# Autodesk Inventor assembly: Rod
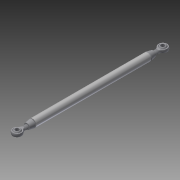
[picture p0: Inventor's stored thumbnail of the model, 180x180]
Saved by Autodesk Inventor 2015 (Build 190159000, 159)
## iProperties
Created: 2016-04-07
Part Number: Rod
Document SubType Name: Assembly
Designer: Mac
Author: Mac
## Documents named in this file (4)
- C:\Users\Mac\Desktop\MotionBase\CAD\MotionBaseCAD\Real Platform\Rod.iam
- C:\Users\Mac\Desktop\MotionBase\CAD\MotionBaseCAD\Real Platform\Rod.ipt
- C:\Users\Mac\Desktop\MotionBase\CAD\MotionBaseCAD\Real Platform\BallJoint.ipt
- C:\Users\Mac\Desktop\MotionBase\CAD\MotionBaseCAD\Real Platform\ThreadedCaps.ipt
## Components (5 placed, 3 different names)
1. Rod:1 — Mate:10, Mate:11, Flush:1, Mate:12, Mate:13, Mate:16, Mate:17
2. BallJoint:1 — Mate:14, Mate:18, Flush:2, Angle:1
3. ThreadedCaps:1 — Mate:13, Mate:14, Mate:17, Mate:18
4. BallJoint:2 — Mate:15, Mate:19, Flush:2
5. ThreadedCaps:2 — Mate:12, Mate:15, Mate:16, Mate:19
## Relationships (13: Mate 10, Flush 2, Angle 1)
- Mate:10: Rod:1
- Mate:11: Rod:1
- Flush:1: Rod:1
- Mate:12: Rod:1 ↔ ThreadedCaps:2
- Mate:13: Rod:1 ↔ ThreadedCaps:1
- Mate:14: BallJoint:1 ↔ ThreadedCaps:1
- Mate:15: BallJoint:2 ↔ ThreadedCaps:2
- Mate:16: Rod:1 ↔ ThreadedCaps:2
- Mate:17: Rod:1 ↔ ThreadedCaps:1
- Mate:18 (-25.4 mm): BallJoint:1 ↔ ThreadedCaps:1
- Mate:19 (-25.4 mm): BallJoint:2 ↔ ThreadedCaps:2
- Flush:2: BallJoint:1 ↔ BallJoint:2
- Angle:1 (0 deg): BallJoint:1
